# Autodesk Inventor assembly: 足ユニット_MIR
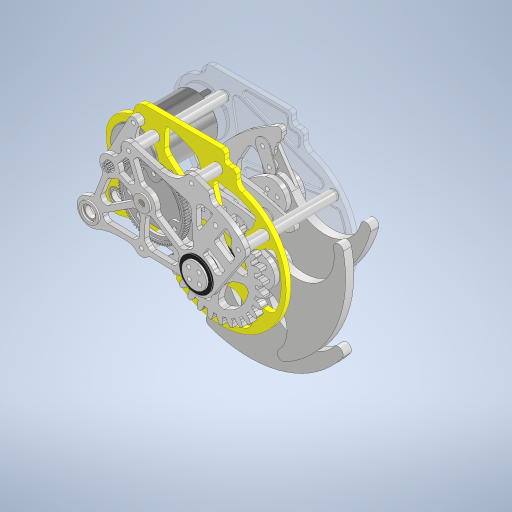
[picture p0: Inventor's stored thumbnail of the model, 512x512]
Saved by Autodesk Inventor 2023 (Build 270158000, 158)
## iProperties
Created: 2022-01-10
Part Number: 足ユニット_MIR
Document SubType Name: Assembly
Designer: muzho
Author: acps
## Documents named in this file (21)
- C:\Users\muzho\Documents\srdc\srdc_2\脚\ミラー\足ユニット_MIR.iam
- C:\Users\muzho\Documents\srdc\srdc_2\スペーサ\l40.ipt
- C:\Users\muzho\Documents\srdc\srdc_2\カム\カム4.ipt
- C:\Users\muzho\Documents\srdc\srdc_2\オイレス\w5f15-17n.ipt
- C:\Users\muzho\Documents\srdc\srdc_2\モータ\M-RS-380.ipt
- C:\Users\muzho\Documents\srdc\srdc_2\ベアリング\φ6φ12ベアリングa.ipt
- C:\Users\muzho\Documents\srdc\srdc_2\脚\ミラー\モータマウント_MIR.ipt
- C:\Users\muzho\Documents\srdc\srdc_2\脚\ミラー\ぴにょん_MIR.ipt
- C:\Users\muzho\Documents\srdc\srdc_2\ベアリング\M-φ4φ8a.ipt
- C:\Users\muzho\Documents\srdc\srdc_2\脚\ギア\初段_多段ギア.iam
- C:\Users\muzho\Documents\srdc\srdc_2\ベアリング\φ4φ8ベアリングa.ipt
- C:\Users\muzho\Documents\srdc\srdc_2\脚\ギア\最終段m2z28t4.ipt
- C:\Users\muzho\Documents\srdc\srdc_2\脚\ミラー\クランク_MIR.iam
- C:\Users\muzho\Documents\srdc\srdc_2\脚\ミラー\揺動節+ヘッケン_MIR.iam
- C:\Users\muzho\Documents\srdc\srdc_2\スペーサ\l14.ipt
- C:\Users\muzho\Documents\srdc\srdc_2\脚\ミラー\足外フレーム_MIR.ipt
- C:\Users\muzho\Documents\srdc\srdc_2\脚\ミラー\ギア抑え_MIR.ipt
- C:\Users\muzho\Documents\srdc\srdc_2\脚\ミラー\足内フレーム_MIR.ipt
- C:\Users\muzho\Documents\srdc\srdc_2\ベアリング\φ6φ10ベアリングa.ipt
- C:\Users\muzho\Documents\srdc\srdc_2\ピン\φ4l20.ipt
- C:\Users\muzho\Documents\srdc\srdc_2\オイレス\w6f15-17a.ipt
## Components (31 placed, 20 different names)
1. l40:1 — 挿入:68, 挿入:89
2. l40:2 — 挿入:67
3. l40:3 — メイト:51, メイト:53, メイト:55, メイト:49, 挿入:65, メイト:64
4. カム4:1 — 挿入:9, 挿入:75, メイト:70, メイト:69, メイト:68, 挿入:51
5. w5f15-17n:1 — 挿入:9
6. M-RS-380:1 — メイト:71, メイト:61, 挿入:31, 挿入:32, メイト:38, メイト:62
7. φ6φ12ベアリングa:1 — 挿入:90, 挿入:86
8. モータマウント_MIR:1 — メイト:71, メイト:61, 挿入:31, メイト:76, 挿入:83
9. ぴにょん_MIR:1 — 挿入:32, メイト:38
10. M-φ4φ8a:1 — メイト:41, 挿入:87, メイト:77
11. 初段_多段ギア:1 [sub-assembly] — メイト:62, メイト:41
12. φ4φ8ベアリングa:1
13. 最終段m2z28t4:1 — 挿入:75, メイト:70, メイト:69, 挿入:88, メイト:79, メイト:78
14. クランク_MIR:1 [sub-assembly] — 挿入:90, メイト:68, 挿入:51, 挿入:54, メイト:52, 挿入:55, メイト:54, 挿入:56, メイト:56, 挿入:52, メイト:50
15. 揺動節+ヘッケン_MIR:1 [sub-assembly] — 挿入:54, メイト:52, メイト:51
16. 揺動節+ヘッケン_MIR:2 [sub-assembly] — 挿入:55, メイト:54, メイト:53
17. 揺動節+ヘッケン_MIR:3 [sub-assembly] — 挿入:56, メイト:56, メイト:55
18. 揺動節+ヘッケン_MIR:4 [sub-assembly] — 挿入:52, メイト:50, メイト:49
19. l14:1
20. l14:2 — 挿入:82
21. l14:3 — 挿入:96, 挿入:93
22. 足外フレーム_MIR:1 — 挿入:86, 挿入:68, 挿入:67, 挿入:65, メイト:64, メイト:75, メイト:74
23. ギア抑え_MIR:1 — 挿入:96, メイト:84
24. 足内フレーム_MIR:1 — 挿入:93, 挿入:89, メイト:76, 挿入:83, 挿入:82, メイト:75, メイト:74, 挿入:85, 挿入:95
25. φ6φ10ベアリングa:1
26. φ6φ10ベアリングa:2 — 挿入:85
27. φ4l20:1 — 挿入:87, メイト:77
28. カム4:2 — 挿入:88, メイト:79, メイト:78, 挿入:92, メイト:83, メイト:82
29. w6f15-17a:1
30. カム4:3 — 挿入:92, メイト:83, メイト:82
31. l14:4 — メイト:84, 挿入:95
## Relationships (50: Mate 26, Insert 24)
- 挿入:9 [Insert]: カム4:1 ↔ w5f15-17n:1
- メイト:71 [Mate]: M-RS-380:1 ↔ モータマウント_MIR:1
- メイト:61 [Mate]: M-RS-380:1 ↔ モータマウント_MIR:1
- 挿入:31 [Insert]: M-RS-380:1 ↔ モータマウント_MIR:1
- 挿入:32 [Insert]: M-RS-380:1 ↔ ぴにょん_MIR:1
- メイト:38 [Mate]: M-RS-380:1 ↔ ぴにょん_MIR:1
- メイト:62 [Mate] (0.3 mm): M-RS-380:1 ↔ 初段_多段ギア:1
- メイト:41 [Mate]: M-φ4φ8a:1 ↔ 初段_多段ギア:1
- 挿入:75 [Insert]: カム4:1 ↔ 最終段m2z28t4:1
- メイト:70 [Mate]: カム4:1 ↔ 最終段m2z28t4:1
- メイト:69 [Mate]: カム4:1 ↔ 最終段m2z28t4:1
- 挿入:90 [Insert]: φ6φ12ベアリングa:1 ↔ クランク_MIR:1
- メイト:68 [Mate]: カム4:1 ↔ クランク_MIR:1
- 挿入:51 [Insert]: カム4:1 ↔ クランク_MIR:1
- 挿入:54 [Insert] (0.25 mm): クランク_MIR:1 ↔ 揺動節+ヘッケン_MIR:1
- メイト:52 [Mate]: クランク_MIR:1 ↔ 揺動節+ヘッケン_MIR:1
- メイト:51 [Mate]: l40:3 ↔ 揺動節+ヘッケン_MIR:1
- 挿入:55 [Insert] (0.25 mm): クランク_MIR:1 ↔ 揺動節+ヘッケン_MIR:2
- メイト:54 [Mate]: クランク_MIR:1 ↔ 揺動節+ヘッケン_MIR:2
- メイト:53 [Mate]: l40:3 ↔ 揺動節+ヘッケン_MIR:2
- 挿入:56 [Insert] (0.25 mm): クランク_MIR:1 ↔ 揺動節+ヘッケン_MIR:3
- メイト:56 [Mate]: クランク_MIR:1 ↔ 揺動節+ヘッケン_MIR:3
- メイト:55 [Mate]: l40:3 ↔ 揺動節+ヘッケン_MIR:3
- 挿入:52 [Insert] (0.25 mm): クランク_MIR:1 ↔ 揺動節+ヘッケン_MIR:4
- メイト:50 [Mate]: クランク_MIR:1 ↔ 揺動節+ヘッケン_MIR:4
- メイト:49 [Mate]: l40:3 ↔ 揺動節+ヘッケン_MIR:4
- 挿入:86 [Insert]: φ6φ12ベアリングa:1 ↔ 足外フレーム_MIR:1
- 挿入:68 [Insert]: l40:1 ↔ 足外フレーム_MIR:1
- 挿入:67 [Insert]: l40:2 ↔ 足外フレーム_MIR:1
- 挿入:65 [Insert]: l40:3 ↔ 足外フレーム_MIR:1
- メイト:64 [Mate]: l40:3 ↔ 足外フレーム_MIR:1
- 挿入:96 [Insert]: l14:3 ↔ ギア抑え_MIR:1
- 挿入:93 [Insert]: l14:3 ↔ 足内フレーム_MIR:1
- 挿入:89 [Insert]: l40:1 ↔ 足内フレーム_MIR:1
- メイト:76 [Mate]: モータマウント_MIR:1 ↔ 足内フレーム_MIR:1
- 挿入:83 [Insert]: モータマウント_MIR:1 ↔ 足内フレーム_MIR:1
- 挿入:82 [Insert]: l14:2 ↔ 足内フレーム_MIR:1
- メイト:75 [Mate]: 足外フレーム_MIR:1 ↔ 足内フレーム_MIR:1
- メイト:74 [Mate]: 足外フレーム_MIR:1 ↔ 足内フレーム_MIR:1
- 挿入:85 [Insert]: 足内フレーム_MIR:1 ↔ φ6φ10ベアリングa:2
- 挿入:87 [Insert] (0.5 mm): M-φ4φ8a:1 ↔ φ4l20:1
- メイト:77 [Mate]: M-φ4φ8a:1 ↔ φ4l20:1
- 挿入:88 [Insert]: 最終段m2z28t4:1 ↔ カム4:2
- メイト:79 [Mate]: 最終段m2z28t4:1 ↔ カム4:2
- メイト:78 [Mate]: 最終段m2z28t4:1 ↔ カム4:2
- 挿入:92 [Insert]: カム4:2 ↔ カム4:3
- メイト:83 [Mate]: カム4:2 ↔ カム4:3
- メイト:82 [Mate]: カム4:2 ↔ カム4:3
- メイト:84 [Mate]: ギア抑え_MIR:1 ↔ l14:4
- 挿入:95 [Insert]: 足内フレーム_MIR:1 ↔ l14:4
